# Autodesk Inventor assembly: ensamblaje nuevo modelo 50 mm mas grande
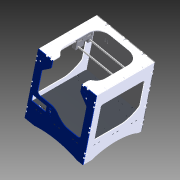
[picture p0: Inventor's stored thumbnail of the model, 180x180]
Saved by Autodesk Inventor 2012 (Build 160160000, 160)
## iProperties
Created: 2014-12-15
Part Number: ensamblaje nuevo modelo 50 mm mas grande
Document SubType Name: Assembly
Designer: PRINCIPAL
Author: PRINCIPAL
## Documents named in this file (10)
- \\LASERROUTERCNC\Users\Laser router cnc\Desktop\compartir con principal\impresora juan marc albert\Ultima modificacio Impresora\modificacio chasis 1-9-14\ensamblaje nuevo modelo 50 mm mas grande.iam
- \\LASERROUTERCNC\Users\Laser router cnc\Desktop\compartir con principal\impresora juan marc albert\Ultima modificacio Impresora\modificacio chasis 1-9-14\base.ipt
- \\LASERROUTERCNC\Users\Laser router cnc\Desktop\compartir con principal\impresora juan marc albert\Ultima modificacio Impresora\modificacio chasis 1-9-14\sostre.ipt
- \\LASERROUTERCNC\Users\Laser router cnc\Desktop\compartir con principal\impresora juan marc albert\Ultima modificacio Impresora\modificacio chasis 1-9-14\esquena.ipt
- \\LASERROUTERCNC\Users\Laser router cnc\Desktop\compartir con principal\impresora juan marc albert\Ultima modificacio Impresora\modificacio chasis 1-9-14\lateral dret.ipt
- \\LASERROUTERCNC\Users\Laser router cnc\Desktop\compartir con principal\impresora juan marc albert\Ultima modificacio Impresora\modificacio chasis 1-9-14\pieza frontal nueva.ipt
- \\LASERROUTERCNC\Users\Laser router cnc\Desktop\compartir con principal\impresora juan marc albert\Ultima modificacio Impresora\modificacio chasis 1-9-14\lateral esquerra.ipt
- \\LASERROUTERCNC\Users\Laser router cnc\Desktop\compartir con principal\impresora juan marc albert\Ultima modificacio Impresora\modificacio chasis 1-9-14\pieza protectora ramps.ipt
- \\LASERROUTERCNC\Users\Laser router cnc\Desktop\compartir con principal\impresora juan marc albert\Ultima modificacio Impresora\modificacio chasis 1-9-14\pieza protectora 2.ipt
- \\LASERROUTERCNC\Users\Laser router cnc\Desktop\compartir con principal\impresora juan marc albert\montaje carro  extrusor.iam
## Components (9 placed, 9 different names)
1. base:1 — Nivelación:15, Coincidencia:8, Coincidencia:9, Nivelación:16, Coincidencia:10, Coincidencia:11
2. sostre:1 — Nivelación:19, Coincidencia:13, Nivelación:20, Nivelación:23, Ángulo:1
3. esquena:1 — Nivelación:21, Nivelación:22, Nivelación:23
4. lateral dret:1 — Nivelación:15, Coincidencia:8, Coincidencia:9, Nivelación:21, Nivelación:22
5. pieza frontal nueva:1 — Nivelación:17, Coincidencia:12, Nivelación:18, Nivelación:19, Coincidencia:13, Nivelación:20, Insertar:7
6. lateral esquerra:1 — Nivelación:11, Coincidencia:5, Coincidencia:6, Nivelación:16, Coincidencia:10, Coincidencia:11, Nivelación:17, Coincidencia:12, Nivelación:18
7. pieza protectora ramps:1 — Nivelación:11, Coincidencia:5, Coincidencia:6, Coincidencia:7, Nivelación:13, Nivelación:14
8. pieza protectora 2:1 — Coincidencia:7, Nivelación:13, Nivelación:14
9. montaje carro  extrusor:1 [sub-assembly] — Insertar:7, Ángulo:1
## Relationships (23: Flush 12, Mate 9, Insert 1, Angle 1)
- Nivelación:11 [Flush]: lateral esquerra:1 ↔ pieza protectora ramps:1
- Coincidencia:5 [Mate]: lateral esquerra:1 ↔ pieza protectora ramps:1
- Coincidencia:6 [Mate]: lateral esquerra:1 ↔ pieza protectora ramps:1
- Coincidencia:7 [Mate]: pieza protectora ramps:1 ↔ pieza protectora 2:1
- Nivelación:13 [Flush]: pieza protectora ramps:1 ↔ pieza protectora 2:1
- Nivelación:14 [Flush] (2.5 mm): pieza protectora ramps:1 ↔ pieza protectora 2:1
- Nivelación:15 [Flush]: base:1 ↔ lateral dret:1
- Coincidencia:8 [Mate]: base:1 ↔ lateral dret:1
- Coincidencia:9 [Mate]: base:1 ↔ lateral dret:1
- Nivelación:16 [Flush]: base:1 ↔ lateral esquerra:1
- Coincidencia:10 [Mate]: base:1 ↔ lateral esquerra:1
- Coincidencia:11 [Mate]: base:1 ↔ lateral esquerra:1
- Nivelación:17 [Flush]: pieza frontal nueva:1 ↔ lateral esquerra:1
- Coincidencia:12 [Mate]: pieza frontal nueva:1 ↔ lateral esquerra:1
- Nivelación:18 [Flush]: pieza frontal nueva:1 ↔ lateral esquerra:1
- Nivelación:19 [Flush]: sostre:1 ↔ pieza frontal nueva:1
- Coincidencia:13 [Mate]: sostre:1 ↔ pieza frontal nueva:1
- Nivelación:20 [Flush]: sostre:1 ↔ pieza frontal nueva:1
- Nivelación:21 [Flush]: esquena:1 ↔ lateral dret:1
- Nivelación:22 [Flush]: esquena:1 ↔ lateral dret:1
- Nivelación:23 [Flush]: sostre:1 ↔ esquena:1
- Insertar:7: pieza frontal nueva:1 ↔ montaje carro  extrusor:1
- Ángulo:1 [Angle] (0 deg): sostre:1 ↔ montaje carro  extrusor:1
